# Autodesk Inventor assembly: Assembly1
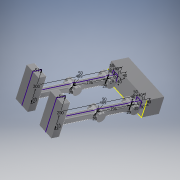
[picture p0: Inventor's stored thumbnail of the model, 180x180]
Saved by Autodesk Inventor 2019 (Build 230136000, 136)
## iProperties
Created: 2022-07-24
Part Number: Assembly1
Document SubType Name: Assembly
Designer: abdul
Author: abdul
## Documents named in this file (3)
- C:\Users\abdul\Desktop\Inventor\Assembly1.iam
- C:\Users\abdul\Desktop\Inventor\for trainig 1.ipt
- C:\Users\abdul\Desktop\Inventor\for trainig 4.ipt
## Components (3 placed, 2 different names)
1. for trainig 1:1 — Rigid:1
2. for trainig 1:2 — Rigid:2, Rigid:3
3. for trainig 4:1 — Rigid:1, Rigid:2, Rigid:3
## Relationships (3: WeldJoint 3)
- Rigid:1 [WeldJoint]: for trainig 1:1 ↔ for trainig 4:1
- Rigid:2 [WeldJoint]: for trainig 1:2 ↔ for trainig 4:1
- Rigid:3 [WeldJoint]: for trainig 1:2 ↔ for trainig 4:1
